# Autodesk Inventor assembly: bett_V3_teil1_sitzbank
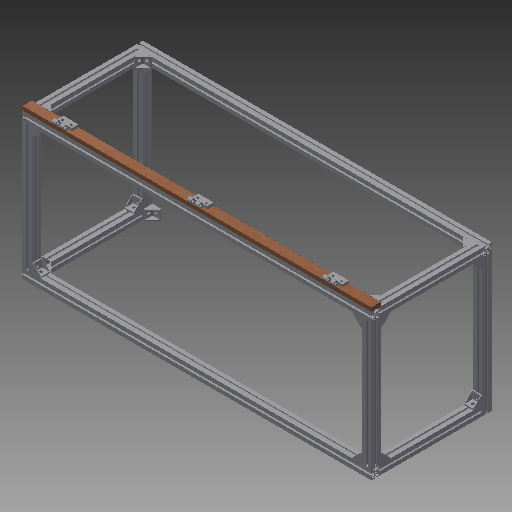
[picture p0: Inventor's stored thumbnail of the model, 512x512]
Saved by Autodesk Inventor 2018 (Build 220112000, 112)
## iProperties
Created: 2020-03-29
Part Number: bett_V3_teil1_sitzbank
Material: Generisch
Document SubType Name: Assembly
Designer: wepet
Mass: 3.22075 g
Surface Area: 205.27 cm^2
Volume: 3.39895 cm^3
Density: 0.947572 g/cm^3
Author: wepet
## Documents named in this file (8)
- C:\Users\wepet\Downloads\anhaenger\current\details\bett\bett_V3\bett_V3_teil1_sitzbank.iam
- C:\Users\wepet\Downloads\anhaenger\current\details\bett\details\item_30x30_40cm.ipt
- C:\Users\wepet\Downloads\anhaenger\current\details\bett\details\item_winkel.ipt
- C:\Users\wepet\Downloads\anhaenger\current\details\bett\details\item_30x30_43cm.ipt
- C:\Users\wepet\Downloads\anhaenger\current\details\bett\details\item_30x30_110cm.ipt
- C:\Users\wepet\Downloads\anhaenger\current\details\bett\details\item_30x30_32cm.ipt
- C:\Users\wepet\Downloads\anhaenger\current\details\bett\bett_V3\bett_V3_detail_deckplatte_scharnier.ipt
- C:\Users\wepet\Downloads\anhaenger\current\details\bett\details\item_scharnier_2_teil.ipt
## Components (37 placed, 7 different names)
1. item_30x30_32cm:1 — Fluchtend:2, Passend:3, Fluchtend:3, Passend:27
2. item_30x30_40cm:1 — Fluchtend:4, Passend:4, Fluchtend:5, Passend:6, Fluchtend:15, Fluchtend:69, Passend:25, Fluchtend:149, Passend:40
3. item_30x30_110cm:1 — Passend:1, Passend:2, Fluchtend:1, Fluchtend:2, Passend:3, Fluchtend:3, Fluchtend:4, Passend:4, Fluchtend:5, Fluchtend:8, Fluchtend:9, Fluchtend:10, Fluchtend:93, Fluchtend:176, Passend:49, Fluchtend:185, Passend:62, Passend:68
4. item_30x30_110cm:3 — Fluchtend:8, Fluchtend:9, Passend:6, Fluchtend:11, Fluchtend:16, Passend:8, Fluchtend:23, Fluchtend:25, Passend:31, Fluchtend:122, Passend:66, Passend:71, Fluchtend:197, Fluchtend:198
5. item_30x30_110cm:2 — Fluchtend:10, Fluchtend:11, Fluchtend:24, Fluchtend:82, Passend:38, Passend:44, Fluchtend:181, Fluchtend:182, Passend:56, Passend:67, Passend:69
6. item_30x30_43cm:1 — Passend:26, Passend:34, Fluchtend:182, Fluchtend:183, Passend:56, Passend:58, Fluchtend:187, Passend:63, Fluchtend:191, Fluchtend:194
7. item_30x30_32cm:2 — Fluchtend:15, Fluchtend:16, Passend:8, Passend:28, Fluchtend:183
8. item_30x30_32cm:3 — Fluchtend:20, Fluchtend:22, Passend:12, Passend:20, Fluchtend:185, Passend:59, Fluchtend:193
9. item_30x30_40cm:3 — Fluchtend:19, Fluchtend:21, Passend:12, Fluchtend:25, Fluchtend:71, Passend:17, Fluchtend:175, Fluchtend:179, Passend:60, Passend:70
10. item_30x30_43cm:3 — Fluchtend:18, Fluchtend:21, Passend:9, Passend:10, Passend:19, Fluchtend:181, Passend:61, Fluchtend:186, Passend:65, Fluchtend:195
11. item_30x30_32cm:4 — Fluchtend:18, Fluchtend:19, Fluchtend:20, Fluchtend:22, Passend:9, Passend:10, Fluchtend:23, Fluchtend:24, Passend:18, Passend:29, Fluchtend:196
12. item_winkel:9 — Fluchtend:71
13. item_winkel:10 — Passend:20
14. item_winkel:11 — Passend:17, Passend:18
15. item_winkel:12 — Passend:19
16. item_winkel:13 — Passend:26, Passend:27
17. item_winkel:14 — Passend:25
18. item_winkel:15 — Fluchtend:69, Passend:28
19. item_winkel:16
20. item_winkel:19 — Passend:29, Passend:31, Fluchtend:94, Passend:70, Fluchtend:196
21. item_winkel:20 — Fluchtend:82, Passend:69
22. item_winkel:23 — Fluchtend:93, Fluchtend:94, Passend:59
23. item_winkel:25 — Passend:58
24. item_winkel:26 — Fluchtend:122, Passend:34, Passend:66
25. item_winkel:30 — Fluchtend:176, Passend:49
26. item_winkel:34 — Fluchtend:187, Passend:67
27. item_winkel:37 — Fluchtend:149, Passend:40, Passend:68
28. item_winkel:38 — Passend:38
29. item_winkel:43 — Passend:44, Passend:61, Fluchtend:186
30. item_winkel:47 — Fluchtend:175
31. item_winkel:48 — Fluchtend:179, Passend:60, Passend:62
32. item_winkel:49 — Passend:65, Fluchtend:193, Fluchtend:195
33. item_winkel:51 — Passend:63, Fluchtend:191, Fluchtend:194
34. bett_V3_detail_deckplatte_scharnier:1 — Passend:71, Fluchtend:197, Fluchtend:198, Passend:72, Passend:73, Passend:74, Passend:75, Passend:76, Passend:77, Fluchtend:199, Fluchtend:200, Fluchtend:201
35. item_scharnier_2_teil:1 — Passend:72, Passend:77, Fluchtend:201
36. item_scharnier_2_teil:2 — Passend:73, Passend:76, Fluchtend:199
37. item_scharnier_2_teil:3 — Passend:74, Passend:75, Fluchtend:200
## Relationships (121: Flush 77, Mate 44)
- Passend:1 [Mate]: item_30x30_110cm:1
- Passend:2 [Mate]: item_30x30_110cm:1
- Fluchtend:1 [Flush]: item_30x30_110cm:1
- Fluchtend:2 [Flush]: item_30x30_32cm:1 ↔ item_30x30_110cm:1
- Passend:3 [Mate]: item_30x30_32cm:1 ↔ item_30x30_110cm:1
- Fluchtend:3 [Flush]: item_30x30_32cm:1 ↔ item_30x30_110cm:1
- Fluchtend:4 [Flush]: item_30x30_40cm:1 ↔ item_30x30_110cm:1
- Passend:4 [Mate]: item_30x30_40cm:1 ↔ item_30x30_110cm:1
- Fluchtend:5 [Flush]: item_30x30_40cm:1 ↔ item_30x30_110cm:1
- Fluchtend:8 [Flush]: item_30x30_110cm:1 ↔ item_30x30_110cm:3
- Fluchtend:9 [Flush]: item_30x30_110cm:1 ↔ item_30x30_110cm:3
- Passend:6 [Mate]: item_30x30_40cm:1 ↔ item_30x30_110cm:3
- Fluchtend:10 [Flush]: item_30x30_110cm:1 ↔ item_30x30_110cm:2
- Fluchtend:11 [Flush]: item_30x30_110cm:3 ↔ item_30x30_110cm:2
- Fluchtend:15 [Flush]: item_30x30_40cm:1 ↔ item_30x30_32cm:2
- Fluchtend:16 [Flush]: item_30x30_110cm:3 ↔ item_30x30_32cm:2
- Passend:8 [Mate]: item_30x30_110cm:3 ↔ item_30x30_32cm:2
- [Flush]: item_30x30_40cm:3 ↔ item_30x30_32cm:4
- Fluchtend:18 [Flush]: item_30x30_43cm:3 ↔ item_30x30_32cm:4
- Fluchtend:19 [Flush]: item_30x30_40cm:3 ↔ item_30x30_32cm:4
- Fluchtend:20 [Flush]: item_30x30_32cm:3 ↔ item_30x30_32cm:4
- Fluchtend:21 [Flush]: item_30x30_40cm:3 ↔ item_30x30_43cm:3
- Fluchtend:22 [Flush]: item_30x30_32cm:3 ↔ item_30x30_32cm:4
- Passend:9 [Mate]: item_30x30_43cm:3 ↔ item_30x30_32cm:4
- Passend:10 [Mate]: item_30x30_43cm:3 ↔ item_30x30_32cm:4
- Passend:12 [Mate]: item_30x30_32cm:3 ↔ item_30x30_40cm:3
- Fluchtend:23 [Flush]: item_30x30_110cm:3 ↔ item_30x30_32cm:4
- Fluchtend:24 [Flush]: item_30x30_110cm:2 ↔ item_30x30_32cm:4
- Fluchtend:25 [Flush]: item_30x30_110cm:3 ↔ item_30x30_40cm:3
- [Flush]: item_winkel:9 ↔ item_winkel:12
- [Flush]: item_winkel:9 ↔ item_winkel:11
- [Flush]: item_winkel:9 ↔ item_winkel:10
- [Flush]: item_winkel:9 ↔ item_winkel:10
- [Flush]: item_winkel:9 ↔ item_winkel:12
- [Flush]: item_winkel:9 ↔ item_winkel:11
- [Flush]: item_winkel:9 ↔ item_winkel:12
- [Flush]: item_winkel:11 ↔ item_winkel:12
- [Flush]: item_winkel:10 ↔ item_winkel:11
- [Flush]: item_winkel:9 ↔ item_winkel:10
- [Flush]: item_winkel:13 ↔ item_winkel:16
- [Flush]: item_winkel:13 ↔ item_winkel:15
- [Flush]: item_winkel:13 ↔ item_winkel:14
- [Flush]: item_winkel:13 ↔ item_winkel:14
- [Flush]: item_winkel:13 ↔ item_winkel:16
- [Flush]: item_winkel:13 ↔ item_winkel:15
- [Flush]: item_winkel:13 ↔ item_winkel:16
- [Flush]: item_winkel:15 ↔ item_winkel:16
- [Flush]: item_winkel:14 ↔ item_winkel:15
- [Flush]: item_winkel:13 ↔ item_winkel:14
- Fluchtend:69 [Flush]: item_30x30_40cm:1 ↔ item_winkel:15
- Fluchtend:71 [Flush]: item_30x30_40cm:3 ↔ item_winkel:9
- Passend:17 [Mate]: item_30x30_40cm:3 ↔ item_winkel:11
- Passend:18 [Mate]: item_30x30_32cm:4 ↔ item_winkel:11
- Passend:19 [Mate]: item_30x30_43cm:3 ↔ item_winkel:12
- Passend:20 [Mate]: item_30x30_32cm:3 ↔ item_winkel:10
- Passend:25 [Mate]: item_30x30_40cm:1 ↔ item_winkel:14
- Passend:26 [Mate]: item_30x30_43cm:1 ↔ item_winkel:13
- Passend:27 [Mate]: item_30x30_32cm:1 ↔ item_winkel:13
- Passend:28 [Mate]: item_30x30_32cm:2 ↔ item_winkel:15
- [Flush]: item_winkel:19 ↔ item_winkel:20
- Passend:29 [Mate]: item_30x30_32cm:4 ↔ item_winkel:19
- Passend:31 [Mate]: item_30x30_110cm:3 ↔ item_winkel:19
- Fluchtend:82 [Flush]: item_30x30_110cm:2 ↔ item_winkel:20
- Fluchtend:93 [Flush]: item_30x30_110cm:1 ↔ item_winkel:23
- Fluchtend:94 [Flush]: item_winkel:19 ↔ item_winkel:23
- [Flush]: item_winkel:25 ↔ item_winkel:26
- [Flush]: item_winkel:25 ↔ item_winkel:26
- [Flush]: item_winkel:25 ↔ item_winkel:26
- [Flush]: item_winkel:26 ↔ item_winkel:30
- Fluchtend:122 [Flush]: item_30x30_110cm:3 ↔ item_winkel:26
- Passend:34 [Mate]: item_30x30_43cm:1 ↔ item_winkel:26
- [Flush]: item_winkel:37 ↔ item_winkel:38
- [Flush]: item_winkel:37 ↔ item_winkel:38
- [Flush]: item_winkel:37 ↔ item_winkel:38
- [Flush]: item_winkel:34 ↔ item_winkel:38
- Passend:38 [Mate]: item_30x30_110cm:2 ↔ item_winkel:38
- Fluchtend:149 [Flush]: item_30x30_40cm:1 ↔ item_winkel:37
- Passend:40 [Mate]: item_30x30_40cm:1 ↔ item_winkel:37
- [Flush]: item_winkel:47 ↔ item_winkel:48
- [Flush]: item_winkel:43 ↔ item_winkel:47
- Passend:44 [Mate]: item_30x30_110cm:2 ↔ item_winkel:43
- Fluchtend:175 [Flush]: item_30x30_40cm:3 ↔ item_winkel:47
- Fluchtend:176 [Flush]: item_30x30_110cm:1 ↔ item_winkel:30
- Passend:49 [Mate]: item_30x30_110cm:1 ↔ item_winkel:30
- Fluchtend:179 [Flush]: item_30x30_40cm:3 ↔ item_winkel:48
- Fluchtend:181 [Flush]: item_30x30_110cm:2 ↔ item_30x30_43cm:3
- Fluchtend:182 [Flush]: item_30x30_110cm:2 ↔ item_30x30_43cm:1
- Fluchtend:183 [Flush]: item_30x30_43cm:1 ↔ item_30x30_32cm:2
- Passend:56 [Mate]: item_30x30_110cm:2 ↔ item_30x30_43cm:1
- Passend:58 [Mate]: item_30x30_43cm:1 ↔ item_winkel:25
- Fluchtend:185 [Flush]: item_30x30_110cm:1 ↔ item_30x30_32cm:3
- Passend:59 [Mate]: item_30x30_32cm:3 ↔ item_winkel:23
- Passend:60 [Mate]: item_30x30_40cm:3 ↔ item_winkel:48
- Passend:61 [Mate]: item_30x30_43cm:3 ↔ item_winkel:43
- Fluchtend:186 [Flush]: item_30x30_43cm:3 ↔ item_winkel:43
- Passend:62 [Mate]: item_30x30_110cm:1 ↔ item_winkel:48
- Fluchtend:187 [Flush]: item_30x30_43cm:1 ↔ item_winkel:34
- Passend:63 [Mate]: item_30x30_43cm:1 ↔ item_winkel:51
- Fluchtend:191 [Flush]: item_30x30_43cm:1 ↔ item_winkel:51
- Passend:65 [Mate]: item_30x30_43cm:3 ↔ item_winkel:49
- Fluchtend:193 [Flush]: item_30x30_32cm:3 ↔ item_winkel:49
- Passend:66 [Mate]: item_30x30_110cm:3 ↔ item_winkel:26
- Passend:67 [Mate]: item_30x30_110cm:2 ↔ item_winkel:34
- Passend:68 [Mate]: item_30x30_110cm:1 ↔ item_winkel:37
- Fluchtend:194 [Flush]: item_30x30_43cm:1 ↔ item_winkel:51
- Fluchtend:195 [Flush]: item_30x30_43cm:3 ↔ item_winkel:49
- Passend:69 [Mate]: item_30x30_110cm:2 ↔ item_winkel:20
- Passend:70 [Mate]: item_30x30_40cm:3 ↔ item_winkel:19
- Fluchtend:196 [Flush]: item_30x30_32cm:4 ↔ item_winkel:19
- Passend:71 [Mate]: item_30x30_110cm:3 ↔ bett_V3_detail_deckplatte_scharnier:1
- Fluchtend:197 [Flush]: item_30x30_110cm:3 ↔ bett_V3_detail_deckplatte_scharnier:1
- Fluchtend:198 [Flush]: item_30x30_110cm:3 ↔ bett_V3_detail_deckplatte_scharnier:1
- Passend:72 [Mate]: bett_V3_detail_deckplatte_scharnier:1 ↔ item_scharnier_2_teil:1
- Passend:73 [Mate]: bett_V3_detail_deckplatte_scharnier:1 ↔ item_scharnier_2_teil:2
- Passend:74 [Mate]: bett_V3_detail_deckplatte_scharnier:1 ↔ item_scharnier_2_teil:3
- Passend:75 [Mate] (-2.9 mm): bett_V3_detail_deckplatte_scharnier:1 ↔ item_scharnier_2_teil:3
- Passend:76 [Mate] (-2.9 mm): bett_V3_detail_deckplatte_scharnier:1 ↔ item_scharnier_2_teil:2
- Passend:77 [Mate] (-2.9 mm): bett_V3_detail_deckplatte_scharnier:1 ↔ item_scharnier_2_teil:1
- Fluchtend:199 [Flush] (10 mm): bett_V3_detail_deckplatte_scharnier:1 ↔ item_scharnier_2_teil:2
- Fluchtend:200 [Flush] (10 mm): bett_V3_detail_deckplatte_scharnier:1 ↔ item_scharnier_2_teil:3
- Fluchtend:201 [Flush] (52.6 mm): bett_V3_detail_deckplatte_scharnier:1 ↔ item_scharnier_2_teil:1
## Named parameters: d24_d21 = 0 mm, d71_d61_d60 = 0 mm, d72_d62_d58 = 0 mm, d73_d63_d59 = 0 mm, d74_d64 = 0 mm, d75_d65 = 0 mm, d76_d66 = 0 mm, d77_d67 = 0 mm, d78_d68 = 0 mm, d79_d69 = 0 mm, d80_d70 = 0 mm, d81_d61_d60 = 0 mm, d82_d62_d58 = 0 mm, d83_d63_d59 = 0 mm, d84_d64 = 0 mm, d85_d65 = 0 mm, d86_d66 = 0 mm, d87_d67 = 0 mm, d88_d68 = 0 mm, d89_d69 = 0 mm, d90_d70 = 0 mm, d113_d68 = 0 mm, d136_d106_d61_d60 = 0 mm, d139_d109_d64 = 0 mm, d145_d115_d70 = 0 mm, d157_d133 = 0 mm, d176_d121_d106_d61_d60 = 0 mm, d179_d124_d109_d64 = 0 mm, d185_d130_d115_d70 = 0 mm, d187_d133 = 0 mm, d213_d183_d128_d113_d68 = 0 mm, d216_d186_d132 = 0 mm
